# Autodesk Inventor assembly: Assembly Plate Assembly
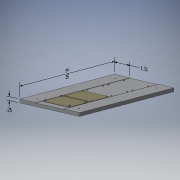
[picture p0: Inventor's stored thumbnail of the model, 180x180]
Saved by Autodesk Inventor 2019.4 (Build 234330000, 330)
## iProperties
Created: 2021-01-11
Part Number: Assembly Plate Assembly
Document SubType Name: Assembly
Designer: caleb
Author: caleb
## Documents named in this file (4)
- C:\Users\cfang\Desktop\nebraska-silicon-lab\Hardware\ETL\Module Assembly\Assembly Plate - boss mounting\Assembly Plate - boss mounting.iam
- C:\Users\cfang\Desktop\nebraska-silicon-lab\Hardware\ETL\Module Assembly\Assembly Plate - boss mounting\Assembly Plate - boss mounting.ipt
- C:\Users\cfang\Desktop\nebraska-silicon-lab\Hardware\ETL\modules\tdr\F10109316--_1-MODULE_ CMS2 ETL_ ALN SUBSTRATE.ipt
- C:\Users\cfang\Desktop\nebraska-silicon-lab\Hardware\ETL\modules\tdr\FC0041908--_1-SHCS_M2x.4x5LGxFT_SS316L_ROLLED_EP.ipt
## Components (7 placed, 3 different names)
1. Assembly Plate - boss mounting:1 — Mate:1, Insert:1, Mate:2, Insert:6
2. F10109316--_1-MODULE_ CMS2 ETL_ ALN SUBSTRATE:1 — Mate:1, Insert:1, Insert:2, Insert:3, Insert:4, Insert:5
3. FC0041908--_1-SHCS_M2x.4x5LGxFT_SS316L_ROLLED_EP:1 — Insert:5
4. FC0041908--_1-SHCS_M2x.4x5LGxFT_SS316L_ROLLED_EP:2 — Insert:4
5. FC0041908--_1-SHCS_M2x.4x5LGxFT_SS316L_ROLLED_EP:3 — Insert:3
6. FC0041908--_1-SHCS_M2x.4x5LGxFT_SS316L_ROLLED_EP:4 — Insert:2
7. F10109316--_1-MODULE_ CMS2 ETL_ ALN SUBSTRATE:2 — Mate:2, Insert:6
## Relationships (8: Insert 6, Mate 2)
- Mate:1: Assembly Plate - boss mounting:1 ↔ F10109316--_1-MODULE_ CMS2 ETL_ ALN SUBSTRATE:1
- Insert:1: Assembly Plate - boss mounting:1 ↔ F10109316--_1-MODULE_ CMS2 ETL_ ALN SUBSTRATE:1
- Insert:2: F10109316--_1-MODULE_ CMS2 ETL_ ALN SUBSTRATE:1 ↔ FC0041908--_1-SHCS_M2x.4x5LGxFT_SS316L_ROLLED_EP:4
- Insert:3: F10109316--_1-MODULE_ CMS2 ETL_ ALN SUBSTRATE:1 ↔ FC0041908--_1-SHCS_M2x.4x5LGxFT_SS316L_ROLLED_EP:3
- Insert:4: F10109316--_1-MODULE_ CMS2 ETL_ ALN SUBSTRATE:1 ↔ FC0041908--_1-SHCS_M2x.4x5LGxFT_SS316L_ROLLED_EP:2
- Insert:5: F10109316--_1-MODULE_ CMS2 ETL_ ALN SUBSTRATE:1 ↔ FC0041908--_1-SHCS_M2x.4x5LGxFT_SS316L_ROLLED_EP:1
- Mate:2: Assembly Plate - boss mounting:1 ↔ F10109316--_1-MODULE_ CMS2 ETL_ ALN SUBSTRATE:2
- Insert:6: Assembly Plate - boss mounting:1 ↔ F10109316--_1-MODULE_ CMS2 ETL_ ALN SUBSTRATE:2
